# Autodesk Inventor assembly: Сборка1
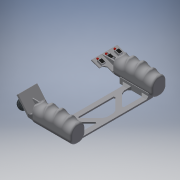
[picture p0: Inventor's stored thumbnail of the model, 180x180]
Saved by Autodesk Inventor 2018 (Build 220112000, 112)
## iProperties
Created: 2019-10-10
Part Number: Сборка1
Material: Типовые
Document SubType Name: Assembly
Designer: Professional
Author: Professional
## Documents named in this file (8)
- C:\Users\Professional\Desktop\Сборка1.iam
- C:\Users\Professional\Desktop\proto_v1.ipt
- C:\Users\Professional\Desktop\forJ.ipt
- C:\Users\Professional\Desktop\JoyStick.ipt
- C:\Users\Professional\Desktop\zenter.ipt
- C:\Users\Professional\Desktop\forB.ipt
- C:\Users\Professional\Desktop\led_3mm.ipt
- C:\Users\Professional\Desktop\btn.ipt
## Components (12 placed, 7 different names)
1. proto_v1:1 — Совмещение:1, Совмещение:2, Совмещение:3, Совмещение:7, Угол:1, Заподлицо:2
2. forJ:1 — Совмещение:1, Совмещение:2, Совмещение:3, Совмещение:4, Совмещение:5, Совмещение:6, Заподлицо:1
3. JoyStick:1 — Совмещение:4, Совмещение:5, Совмещение:6
4. zenter:1 — Совмещение:7, Угол:1, Совмещение:8
5. proto_v1:2 — Совмещение:8, Заподлицо:1, Заподлицо:2, Совмещение:9, Совмещение:10, Совмещение:11
6. forB:1 — Совмещение:9, Совмещение:10, Совмещение:11, Совмещение:12, Совмещение:13, Совмещение:14, Совмещение:15, Совмещение:16, Совмещение:17, Совмещение:18, Совмещение:19, Совмещение:20, Совмещение:21, Совмещение:22, Совмещение:23, Совмещение:24, Совмещение:25, Совмещение:26
7. led_3mm:1 — Совмещение:12, Совмещение:13
8. led_3mm:2 — Совмещение:14, Совмещение:17
9. led_3mm:3 — Совмещение:15, Совмещение:16
10. btn:1 — Совмещение:18, Совмещение:19, Совмещение:20
11. btn:2 — Совмещение:21, Совмещение:25, Совмещение:26
12. btn:3 — Совмещение:22, Совмещение:23, Совмещение:24
## Relationships (29: Mate 26, Flush 2, Angle 1)
- Совмещение:1 [Mate]: proto_v1:1 ↔ forJ:1
- Совмещение:2 [Mate]: proto_v1:1 ↔ forJ:1
- Совмещение:3 [Mate]: proto_v1:1 ↔ forJ:1
- Совмещение:4 [Mate]: forJ:1 ↔ JoyStick:1
- Совмещение:5 [Mate]: forJ:1 ↔ JoyStick:1
- Совмещение:6 [Mate]: forJ:1 ↔ JoyStick:1
- Совмещение:7 [Mate]: proto_v1:1 ↔ zenter:1
- Угол:1 [Angle] (0 deg): proto_v1:1 ↔ zenter:1
- Совмещение:8 [Mate]: zenter:1 ↔ proto_v1:2
- Заподлицо:1 [Flush]: forJ:1 ↔ proto_v1:2
- Заподлицо:2 [Flush]: proto_v1:1 ↔ proto_v1:2
- Совмещение:9 [Mate]: proto_v1:2 ↔ forB:1
- Совмещение:10 [Mate]: proto_v1:2 ↔ forB:1
- Совмещение:11 [Mate]: proto_v1:2 ↔ forB:1
- Совмещение:12 [Mate]: forB:1 ↔ led_3mm:1
- Совмещение:13 [Mate]: forB:1 ↔ led_3mm:1
- Совмещение:14 [Mate]: forB:1 ↔ led_3mm:2
- Совмещение:15 [Mate]: forB:1 ↔ led_3mm:3
- Совмещение:16 [Mate]: forB:1 ↔ led_3mm:3
- Совмещение:17 [Mate]: forB:1 ↔ led_3mm:2
- Совмещение:18 [Mate]: forB:1 ↔ btn:1
- Совмещение:19 [Mate]: forB:1 ↔ btn:1
- Совмещение:20 [Mate]: forB:1 ↔ btn:1
- Совмещение:21 [Mate]: forB:1 ↔ btn:2
- Совмещение:22 [Mate]: forB:1 ↔ btn:3
- Совмещение:23 [Mate]: forB:1 ↔ btn:3
- Совмещение:24 [Mate]: forB:1 ↔ btn:3
- Совмещение:25 [Mate]: forB:1 ↔ btn:2
- Совмещение:26 [Mate]: forB:1 ↔ btn:2
